# Autodesk Inventor assembly: Ensamble Cajas Electrónica
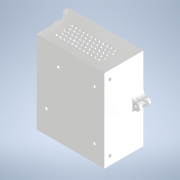
[picture p0: Inventor's stored thumbnail of the model, 180x180]
Saved by Autodesk Inventor 2020.3 (Build 243373000, 373)
## iProperties
Created: 2021-04-10
Part Number: Ensamble Cajas Electrónica
Document SubType Name: Assembly
Designer: juanp
Author: juanp
## Documents named in this file (3)
- C:\Users\juanp\Desktop\Robocol\Cajas Electronica\Ensamble Cajas Electrónica.iam
- C:\Users\juanp\Desktop\Robocol\Cajas Electronica\Main.ipt
- C:\Users\juanp\Desktop\Robocol\Cajas Electronica\Junta.ipt
## Components (2 placed, 2 different names)
1. Main:1 — Mate:4, Mate:2, Mate:3, Flush:2, Mate:5
2. Junta:1 — Mate:4, Mate:5
## Relationships (5: Mate 4, Flush 1)
- Mate:4: Main:1 ↔ Junta:1
- Mate:2: Main:1
- Mate:3: Main:1
- Flush:2: Main:1
- Mate:5: Main:1 ↔ Junta:1
